# Autodesk Inventor assembly: сборка raspberry pi
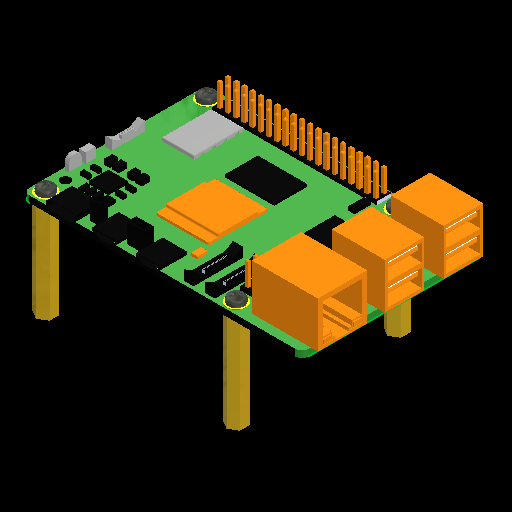
[picture p0: Inventor's stored thumbnail of the model, 512x512]
Saved by Autodesk Inventor 2025 (Build 290162000, 162)
## iProperties
Created: 2025-03-03
Part Number: сборка raspberry pi
Document SubType Name: Assembly
Designer: volko
Mass: 22.9339 g
Surface Area: 47.8076 cm^2
Volume: 2.94092 cm^3
Density: 7.79819 g/cm^3
Author: volko
## Documents named in this file (4)
- C:\Users\volko\Desktop\диплом\Модели\детали\сборка raspberry pi.iam
- C:\Users\volko\Desktop\диплом\Модели\детали\Raspberry Pi 5.ipt
- C:\Users\volko\Desktop\диплом\Модели\детали\втулки крепления электроники.ipt
- C:\Users\volko\Desktop\диплом\Модели\детали\стандартные изделия\ru-RU\ISO 7045  H\ISO 7045 - M2,5 x 8_ - 4.8 - H - ISO.ipt
## Components (9 placed, 3 different names)
1. Raspberry Pi 5:1 — Совмещение:1, Совмещение:2, Совмещение:3, Совмещение:4, Совмещение:5, Совмещение:6, Совмещение:7, Совмещение:8, Совмещение:12, Совмещение:13, Совмещение:14, Заподлицо:1, Заподлицо:2, Заподлицо:3, Совмещение:15, Совмещение:16, Совмещение:17
2. втулки крепления электроники:1 — Совмещение:1, Совмещение:5, Совмещение:9
3. втулки крепления электроники:2 — Совмещение:2, Совмещение:8
4. втулки крепления электроники:3 — Совмещение:3, Совмещение:7
5. втулки крепления электроники:4 — Совмещение:4, Совмещение:6, Совмещение:11
6. ISO 7045 H M2,5 x 8 - 4.8 - H:1 — Совмещение:9, Совмещение:14
7. ISO 7045 H M2,5 x 8 - 4.8 - H:2 — Совмещение:13, Совмещение:17
8. ISO 7045 H M2,5 x 8 - 4.8 - H:3 — Совмещение:11, Совмещение:15
9. ISO 7045 H M2,5 x 8 - 4.8 - H:4 — Совмещение:12, Совмещение:16
## Relationships (19: Mate 16, Flush 3)
- Совмещение:1 [Mate]: Raspberry Pi 5:1 ↔ втулки крепления электроники:1
- Совмещение:2 [Mate]: Raspberry Pi 5:1 ↔ втулки крепления электроники:2
- Совмещение:3 [Mate]: Raspberry Pi 5:1 ↔ втулки крепления электроники:3
- Совмещение:4 [Mate]: Raspberry Pi 5:1 ↔ втулки крепления электроники:4
- Совмещение:5 [Mate]: Raspberry Pi 5:1 ↔ втулки крепления электроники:1
- Совмещение:6 [Mate]: Raspberry Pi 5:1 ↔ втулки крепления электроники:4
- Совмещение:7 [Mate]: Raspberry Pi 5:1 ↔ втулки крепления электроники:3
- Совмещение:8 [Mate]: Raspberry Pi 5:1 ↔ втулки крепления электроники:2
- Совмещение:9 [Mate]: втулки крепления электроники:1 ↔ ISO 7045 H M2,5 x 8 - 4.8 - H:1
- Совмещение:11 [Mate]: втулки крепления электроники:4 ↔ ISO 7045 H M2,5 x 8 - 4.8 - H:3
- Совмещение:12 [Mate]: Raspberry Pi 5:1 ↔ ISO 7045 H M2,5 x 8 - 4.8 - H:4
- Совмещение:13 [Mate]: Raspberry Pi 5:1 ↔ ISO 7045 H M2,5 x 8 - 4.8 - H:2
- Совмещение:14 [Mate]: Raspberry Pi 5:1 ↔ ISO 7045 H M2,5 x 8 - 4.8 - H:1
- Заподлицо:1 [Flush]: Raspberry Pi 5:1
- Заподлицо:2 [Flush]: Raspberry Pi 5:1
- Заподлицо:3 [Flush]: Raspberry Pi 5:1
- Совмещение:15 [Mate]: Raspberry Pi 5:1 ↔ ISO 7045 H M2,5 x 8 - 4.8 - H:3
- Совмещение:16 [Mate]: Raspberry Pi 5:1 ↔ ISO 7045 H M2,5 x 8 - 4.8 - H:4
- Совмещение:17 [Mate]: Raspberry Pi 5:1 ↔ ISO 7045 H M2,5 x 8 - 4.8 - H:2
